# Autodesk Inventor assembly: A2017_T5_02
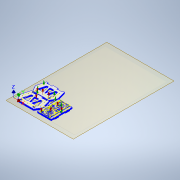
[picture p0: Inventor's stored thumbnail of the model, 180x180]
Saved by Autodesk Inventor 2020 (Build 240168000, 168)
## iProperties
Created: 2021-08-27
Part Number: A2017_T5_02
Document SubType Name: Assembly
Designer: Masato
Author: Masato
## Documents named in this file (4)
- C:\Users\naoki\Documents\Inventor\CitBrains\git_clone\OpenPlatform4_1\コックピット以外\OpenPlatform_ver3_0\cam\A2017_T5_02.iam
- C:\Users\naoki\Documents\Inventor\CitBrains\git_clone\OpenPlatform4_1\コックピット以外\OpenPlatform_ver3_0\cam\Disposable_Board.ipt
- C:\Users\naoki\Documents\Inventor\CitBrains\git_clone\OpenPlatform4_1\コックピット以外\OpenPlatform_ver3_0\UpperBody\Trunk\Trunk_lower_side_frame.ipt
- C:\Users\naoki\Documents\Inventor\CitBrains\git_clone\OpenPlatform4_1\コックピット以外\OpenPlatform_ver3_0\UpperBody\Arm\Shoulder_horn_frame.ipt
## Components (5 placed, 3 different names)
1. Disposable_Board:1 — メイト:2, メイト:1, フラッシュ:1, フラッシュ:2, メイト:4, メイト:5, フラッシュ:3, 正接:1, フラッシュ:4
2. Trunk_lower_side_frame:1 — メイト:4, フラッシュ:3, 正接:1, 正接:2
3. Trunk_lower_side_frame:2
4. Shoulder_horn_frame:1 — メイト:5, フラッシュ:4, 正接:2
5. Shoulder_horn_frame:2
## Component patterns: (2 elements, first: Trunk_lower_side_frame:1), (2 elements, first: Shoulder_horn_frame:1)
## Relationships (10: Mate 4, Flush 4, Tangent 2)
- メイト:2 [Mate]: Disposable_Board:1
- メイト:1 [Mate]: Disposable_Board:1
- フラッシュ:1 [Flush]: Disposable_Board:1
- フラッシュ:2 [Flush]: Disposable_Board:1
- メイト:4 [Mate]: Disposable_Board:1 ↔ Trunk_lower_side_frame:1
- メイト:5 [Mate]: Disposable_Board:1 ↔ Shoulder_horn_frame:1
- フラッシュ:3 [Flush] (2 mm): Disposable_Board:1 ↔ Trunk_lower_side_frame:1
- 正接:1 [Tangent] (2 mm): Disposable_Board:1 ↔ Trunk_lower_side_frame:1
- フラッシュ:4 [Flush] (2 mm): Disposable_Board:1 ↔ Shoulder_horn_frame:1
- 正接:2 [Tangent] (2 mm): Trunk_lower_side_frame:1 ↔ Shoulder_horn_frame:1
